# Autodesk Inventor assembly: EL2-900
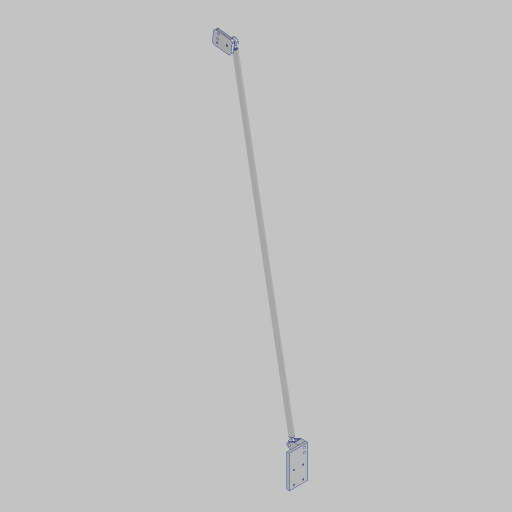
[picture p0: Inventor's stored thumbnail of the model, 512x512]
Saved by Autodesk Inventor 2023.5 (Build 275446000, 446)
## iProperties
Created: 2025-02-12
Part Number: EL2-900
Document SubType Name: Assembly
Designer: slick
Author: slick
## Documents named in this file (6)
- C:\Users\slick\OneDrive\Desktop\2025-ReefScape---CAD\Elevator\EL2\EL2-900.iam
- C:\Users\slick\OneDrive\Desktop\2025-ReefScape---CAD\Elevator\EL2\EL2-025.ipt
- C:\Users\slick\OneDrive\Desktop\2025-ReefScape---CAD\COMMON PARTS\MCMASTER\60645K812_Ball Joint Rod End\60645K812_Ball Joint Rod End.ipt
- C:\Users\slick\OneDrive\Desktop\2025-ReefScape---CAD\Elevator\EL2\EL2-027.ipt
- C:\Users\slick\OneDrive\Desktop\2025-ReefScape---CAD\Elevator\EL2\EL2-026.ipt
- C:\Users\slick\OneDrive\Desktop\2025-ReefScape---CAD\Elevator\EL2\EL2-028.ipt
## Components (6 placed, 5 different names)
1. EL2-025:1 — Mate:1, Mate:2, Mate:3, Mate:4, Mate:8
2. 60645K812_Ball Joint Rod End:1 — Mate:1, Mate:4, Mate:7, Mate:8
3. 60645K812_Ball Joint Rod End:2 — Mate:2, Mate:3, Mate:5, Mate:6
4. EL2-027:1 — Insert:1, Insert:2, Angle:1
5. EL2-026:1 — Insert:1, Insert:2, Mate:5, Mate:6
6. EL2-028:1 — Mate:7, Angle:1
## Relationships (11: Mate 8, Insert 2, Angle 1)
- Mate:1: EL2-025:1 ↔ 60645K812_Ball Joint Rod End:1
- Mate:2: EL2-025:1 ↔ 60645K812_Ball Joint Rod End:2
- Mate:3 (15.875 mm): EL2-025:1 ↔ 60645K812_Ball Joint Rod End:2
- Mate:4 (31.75 mm): EL2-025:1 ↔ 60645K812_Ball Joint Rod End:1
- Insert:1: EL2-027:1 ↔ EL2-026:1
- Insert:2: EL2-027:1 ↔ EL2-026:1
- Mate:5: 60645K812_Ball Joint Rod End:2 ↔ EL2-026:1
- Mate:6 (0.7937 mm): 60645K812_Ball Joint Rod End:2 ↔ EL2-026:1
- Mate:7: 60645K812_Ball Joint Rod End:1 ↔ EL2-028:1
- Angle:1 (0 deg): EL2-027:1 ↔ EL2-028:1
- Mate:8 (15.875 mm): EL2-025:1 ↔ 60645K812_Ball Joint Rod End:1
